# Autodesk Inventor assembly: Chessboard Top
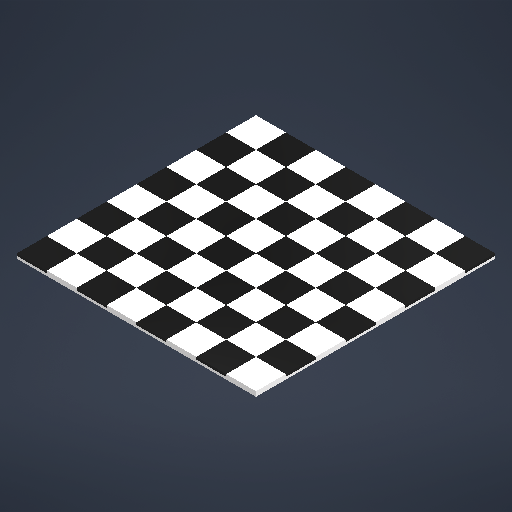
[picture p0: Inventor's stored thumbnail of the model, 512x512]
Saved by Autodesk Inventor 2026 (Build 300175000, 175)
## iProperties
Created: 2025-04-18
Part Number: Chessboard Top
Document SubType Name: Assembly
Designer: ckyiu
Author: ckyiu
## Documents named in this file (5)
- F:\Chessboard-Design\Design\Core\Chessboard Top.iam
- F:\Chessboard-Design\Design\Core\Squares\Square Holder.ipt
- F:\Chessboard-Design\Design\Core\Squares\White Square.ipt
- F:\Chessboard-Design\Design\Core\Squares\Black Square.ipt
- F:\Chessboard-Design\Design\My-Inventor-Parts\Hardware\(9.5mm diameter 1.6mm height) 5862K143_Neodymium Magnet.ipt
## Components (129 placed, 4 different names)
1. Square Holder:1 — Flush:1, Flush:2, Mate:1, Mate:2, Flush:3, Flush:4, Mate:3, Flush:5, Flush:6, Mate:4, Flush:7, Flush:8, Insert:1
2. White Square:1 — Flush:1, Flush:2, Mate:1
3. White Square:2
4. White Square:3
5. White Square:4
6. White Square:5
7. White Square:6
8. White Square:7
9. White Square:8
10. White Square:9
11. White Square:10
12. White Square:11
13. White Square:12
14. White Square:13
15. White Square:14
16. White Square:15
17. White Square:16
18. White Square:17 — Mate:2, Flush:3, Flush:4
19. White Square:18
20. White Square:19
21. White Square:20
22. White Square:21
23. White Square:22
24. White Square:23
25. White Square:24
26. White Square:25
27. White Square:26
28. White Square:27
29. White Square:28
30. White Square:29
31. White Square:30
32. White Square:31
33. White Square:32
34. Black Square:1 — Mate:3, Flush:5, Flush:6
35. Black Square:2
36. Black Square:3
37. Black Square:4
38. Black Square:5
39. Black Square:6
40. Black Square:7
41. Black Square:8
42. Black Square:9
43. Black Square:10
44. Black Square:11
45. Black Square:12
46. Black Square:13
47. Black Square:14
48. Black Square:15
49. Black Square:16
50. Black Square:17 — Mate:4, Flush:7, Flush:8
51. Black Square:18
52. Black Square:19
53. Black Square:20
54. Black Square:21
55. Black Square:22
56. Black Square:23
57. Black Square:24
58. Black Square:25
59. Black Square:26
60. Black Square:27
61. Black Square:28
62. Black Square:29
63. Black Square:30
64. Black Square:31
65. Black Square:32
66. (9.5mm diameter 1.6mm height) 5862K143_Neodymium Magnet:1 — Insert:1
67. (9.5mm diameter 1.6mm height) 5862K143_Neodymium Magnet:2
68. (9.5mm diameter 1.6mm height) 5862K143_Neodymium Magnet:3
69. (9.5mm diameter 1.6mm height) 5862K143_Neodymium Magnet:4
70. (9.5mm diameter 1.6mm height) 5862K143_Neodymium Magnet:5
71. (9.5mm diameter 1.6mm height) 5862K143_Neodymium Magnet:6
72. (9.5mm diameter 1.6mm height) 5862K143_Neodymium Magnet:7
73. (9.5mm diameter 1.6mm height) 5862K143_Neodymium Magnet:8
74. (9.5mm diameter 1.6mm height) 5862K143_Neodymium Magnet:9
75. (9.5mm diameter 1.6mm height) 5862K143_Neodymium Magnet:10
76. (9.5mm diameter 1.6mm height) 5862K143_Neodymium Magnet:11
77. (9.5mm diameter 1.6mm height) 5862K143_Neodymium Magnet:12
78. (9.5mm diameter 1.6mm height) 5862K143_Neodymium Magnet:13
79. (9.5mm diameter 1.6mm height) 5862K143_Neodymium Magnet:14
80. (9.5mm diameter 1.6mm height) 5862K143_Neodymium Magnet:15
81. (9.5mm diameter 1.6mm height) 5862K143_Neodymium Magnet:16
82. (9.5mm diameter 1.6mm height) 5862K143_Neodymium Magnet:17
83. (9.5mm diameter 1.6mm height) 5862K143_Neodymium Magnet:18
84. (9.5mm diameter 1.6mm height) 5862K143_Neodymium Magnet:19
85. (9.5mm diameter 1.6mm height) 5862K143_Neodymium Magnet:20
86. (9.5mm diameter 1.6mm height) 5862K143_Neodymium Magnet:21
87. (9.5mm diameter 1.6mm height) 5862K143_Neodymium Magnet:22
88. (9.5mm diameter 1.6mm height) 5862K143_Neodymium Magnet:23
89. (9.5mm diameter 1.6mm height) 5862K143_Neodymium Magnet:24
90. (9.5mm diameter 1.6mm height) 5862K143_Neodymium Magnet:25
91. (9.5mm diameter 1.6mm height) 5862K143_Neodymium Magnet:26
92. (9.5mm diameter 1.6mm height) 5862K143_Neodymium Magnet:27
93. (9.5mm diameter 1.6mm height) 5862K143_Neodymium Magnet:28
94. (9.5mm diameter 1.6mm height) 5862K143_Neodymium Magnet:29
95. (9.5mm diameter 1.6mm height) 5862K143_Neodymium Magnet:30
96. (9.5mm diameter 1.6mm height) 5862K143_Neodymium Magnet:31
97. (9.5mm diameter 1.6mm height) 5862K143_Neodymium Magnet:32
98. (9.5mm diameter 1.6mm height) 5862K143_Neodymium Magnet:33
99. (9.5mm diameter 1.6mm height) 5862K143_Neodymium Magnet:34
100. (9.5mm diameter 1.6mm height) 5862K143_Neodymium Magnet:35
101. (9.5mm diameter 1.6mm height) 5862K143_Neodymium Magnet:36
102. (9.5mm diameter 1.6mm height) 5862K143_Neodymium Magnet:37
103. (9.5mm diameter 1.6mm height) 5862K143_Neodymium Magnet:38
104. (9.5mm diameter 1.6mm height) 5862K143_Neodymium Magnet:39
105. (9.5mm diameter 1.6mm height) 5862K143_Neodymium Magnet:40
106. (9.5mm diameter 1.6mm height) 5862K143_Neodymium Magnet:41
107. (9.5mm diameter 1.6mm height) 5862K143_Neodymium Magnet:42
108. (9.5mm diameter 1.6mm height) 5862K143_Neodymium Magnet:43
109. (9.5mm diameter 1.6mm height) 5862K143_Neodymium Magnet:44
110. (9.5mm diameter 1.6mm height) 5862K143_Neodymium Magnet:45
111. (9.5mm diameter 1.6mm height) 5862K143_Neodymium Magnet:46
112. (9.5mm diameter 1.6mm height) 5862K143_Neodymium Magnet:47
113. (9.5mm diameter 1.6mm height) 5862K143_Neodymium Magnet:48
114. (9.5mm diameter 1.6mm height) 5862K143_Neodymium Magnet:49
115. (9.5mm diameter 1.6mm height) 5862K143_Neodymium Magnet:50
116. (9.5mm diameter 1.6mm height) 5862K143_Neodymium Magnet:51
117. (9.5mm diameter 1.6mm height) 5862K143_Neodymium Magnet:52
118. (9.5mm diameter 1.6mm height) 5862K143_Neodymium Magnet:53
119. (9.5mm diameter 1.6mm height) 5862K143_Neodymium Magnet:54
120. (9.5mm diameter 1.6mm height) 5862K143_Neodymium Magnet:55
121. (9.5mm diameter 1.6mm height) 5862K143_Neodymium Magnet:56
122. (9.5mm diameter 1.6mm height) 5862K143_Neodymium Magnet:57
123. (9.5mm diameter 1.6mm height) 5862K143_Neodymium Magnet:58
124. (9.5mm diameter 1.6mm height) 5862K143_Neodymium Magnet:59
125. (9.5mm diameter 1.6mm height) 5862K143_Neodymium Magnet:60
126. (9.5mm diameter 1.6mm height) 5862K143_Neodymium Magnet:61
127. (9.5mm diameter 1.6mm height) 5862K143_Neodymium Magnet:62
128. (9.5mm diameter 1.6mm height) 5862K143_Neodymium Magnet:63
129. (9.5mm diameter 1.6mm height) 5862K143_Neodymium Magnet:64
## Component patterns: (16 elements, first: White Square:1), (16 elements, first: White Square:17), (16 elements, first: Black Square:1), (16 elements, first: Black Square:17), (64 elements, first: (9.5mm diameter 1.6mm height) 5862K143_Neodymium Magnet:1)
## Relationships (13: Flush 8, Mate 4, Insert 1)
- Flush:1: Square Holder:1 ↔ White Square:1
- Flush:2: Square Holder:1 ↔ White Square:1
- Mate:1: Square Holder:1 ↔ White Square:1
- Mate:2: Square Holder:1 ↔ White Square:17
- Flush:3: Square Holder:1 ↔ White Square:17
- Flush:4: Square Holder:1 ↔ White Square:17
- Mate:3: Square Holder:1 ↔ Black Square:1
- Flush:5: Square Holder:1 ↔ Black Square:1
- Flush:6: Square Holder:1 ↔ Black Square:1
- Mate:4: Square Holder:1 ↔ Black Square:17
- Flush:7: Square Holder:1 ↔ Black Square:17
- Flush:8: Square Holder:1 ↔ Black Square:17
- Insert:1: Square Holder:1 ↔ (9.5mm diameter 1.6mm height) 5862K143_Neodymium Magnet:1
